# Autodesk Inventor assembly: shooter launcher
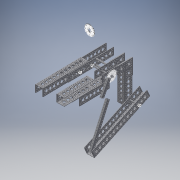
[picture p0: Inventor's stored thumbnail of the model, 180x180]
Saved by Autodesk Inventor 2017 (Build 210142000, 142)
## iProperties
Created: 2018-05-23
Part Number: shooter launcher
Document SubType Name: Assembly
Designer: User
Author: User
## Documents named in this file (16)
- C:\Robotics\CAD\2018-19_CAD\Offseason\shooter launcher.iam
- catapalt ball shoote.iam
- C:\Robotics\CAD\COTSParts\Actobotics\585 parts\585446Channel6in.ipt
- C:\Robotics\CAD\COTSParts\Actobotics\585 parts\585628FlatPattern90degreesA.ipt
- C:\Robotics\CAD\COTSParts\Tetrix\Hex standoff 2in.ipt
- C:\Robotics\CAD\COTSParts\Actobotics\615 parts\615106Sprocket.5inBore.25inPitch24Teeth.ipt
- C:\Robotics\CAD\COTSParts\Actobotics\535 parts\535198Bearing.25ID.5OD.ipt
- C:\Robotics\CAD\COTSParts\Actobotics\Collar.ipt
- C:\Robotics\CAD\COTSParts\Actobotics\585 parts\585450Channel9in.ipt
- C:\Robotics\CAD\COTSParts\Actobotics\585 parts\585454Channel12in.ipt
- C:\Robotics\CAD\COTSParts\Actobotics\634 parts\634080.25inDShaft4inLong.ipt
- C:\Robotics\CAD\COTSParts\Fasteners\Nylon spacer .25.ipt
- C:\Robotics\CAD\COTSParts\Actobotics\545 parts\545618 clamping hub.ipt
- C:\Robotics\CAD\COTSParts\Actobotics\634 parts\634082.25inDShaft6inLong.ipt
- C:\Robotics\CAD\COTSParts\Actobotics\585 parts\585396MiniChannel8in.ipt
- C:\Robotics\CAD\COTSParts\Actobotics\585 parts\585382MiniChannel3in.ipt
## Components (33 placed, 14 different names)
1. 585446Channel6in:1 — Mate:1, Flush:1, Flush:2, Mate:2, Flush:4, Mate:3, Flush:6, Insert:1, Mate:10, Mate:11, Mate:12, Mate:13, Mate:14, Insert:9, Flush:7, Insert:11, Mate:57
2. 585446Channel6in:2 — Mate:1, Flush:1, Flush:2, Flush:3, Flush:5, Mate:26, Mate:27, Mate:28, Mate:29
3. 585628FlatPattern90degreesA:1 — Mate:3, Flush:5, Flush:6
4. 585628FlatPattern90degreesA:2 — Mate:2, Flush:3, Flush:4
5. Hex standoff 2in:1 — Insert:11
6. Hex standoff 2in:3 — Insert:1, Mate:25
7. 615106Sprocket.5inBore.25inPitch24Teeth:1 — Mate:58, Mate:59, Mate:60, Mate:61
8. 615106Sprocket.5inBore.25inPitch24Teeth:2
9. 535198Bearing.25ID.5OD:1 — Insert:10, Mate:21
10. 535198Bearing.25ID.5OD:2 — Mate:12, Mate:13
11. 535198Bearing.25ID.5OD:3 — Mate:10, Mate:11, Insert:6
12. 535198Bearing.25ID.5OD:4 — Insert:8, Mate:23, Mate:54
13. Collar:1 — Insert:6, Mate:20
14. Collar:3 — Mate:21, Mate:55
15. Collar:4 — Insert:8, Mate:53, Flush:11
16. 585446Channel6in:3 — Mate:14, Insert:9, Flush:7, Mate:15, Flush:8, Mate:16
17. 585446Channel6in:4 — Mate:15, Flush:8, Mate:16, Flush:9
18. 585450Channel9in:1 — Mate:17, Mate:19, Mate:20, Insert:10, Mate:23, Flush:9, Mate:24, Mate:25, Mate:54
19. 585450Channel9in:2 — Mate:17, Mate:19, Mate:24
20. 585454Channel12in:1 — Mate:30, Mate:38, Mate:49, Insert:12
21. 634080.25inDShaft4inLong:1 — Mate:39, Mate:40, Mate:44, Mate:46, Mate:51, Flush:10
22. 535198Bearing.25ID.5OD:5 — Mate:38, Mate:48, Mate:51
23. 535198Bearing.25ID.5OD:6 — Mate:28, Mate:29, Mate:52
24. 535198Bearing.25ID.5OD:7 — Mate:30, Mate:40, Mate:49, Mate:50
25. 535198Bearing.25ID.5OD:8 — Mate:26, Mate:27, Mate:35, Mate:47
26. Collar:5 — Mate:35, Mate:39, Mate:50, Flush:10
27. Collar:6 — Mate:44, Mate:52
28. Nylon spacer .25:1 — Mate:46, Mate:47, Mate:48
29. Collar:7
30. 545618 clamping hub:1 — Mate:56, Mate:57, Mate:58, Mate:59, Mate:60
31. 634082.25inDShaft6inLong:1 — Mate:53, Mate:55, Mate:56, Flush:11
32. 585396MiniChannel8in:1 — Insert:12, Mate:62
33. 585382MiniChannel3in:1 — Mate:61, Mate:62
## Relationships (62: Mate 44, Flush 11, Insert 7)
- Mate:1: 585446Channel6in:1 ↔ 585446Channel6in:2
- Flush:1: 585446Channel6in:1 ↔ 585446Channel6in:2
- Flush:2: 585446Channel6in:1 ↔ 585446Channel6in:2
- Mate:2: 585446Channel6in:1 ↔ 585628FlatPattern90degreesA:2
- Flush:3: 585446Channel6in:2 ↔ 585628FlatPattern90degreesA:2
- Flush:4: 585446Channel6in:1 ↔ 585628FlatPattern90degreesA:2
- Mate:3: 585446Channel6in:1 ↔ 585628FlatPattern90degreesA:1
- Flush:5: 585446Channel6in:2 ↔ 585628FlatPattern90degreesA:1
- Flush:6: 585446Channel6in:1 ↔ 585628FlatPattern90degreesA:1
- Insert:1: 585446Channel6in:1 ↔ Hex standoff 2in:3
- Mate:10: 585446Channel6in:1 ↔ 535198Bearing.25ID.5OD:3
- Mate:11: 585446Channel6in:1 ↔ 535198Bearing.25ID.5OD:3
- Mate:12: 585446Channel6in:1 ↔ 535198Bearing.25ID.5OD:2
- Mate:13: 585446Channel6in:1 ↔ 535198Bearing.25ID.5OD:2
- Insert:6: 535198Bearing.25ID.5OD:3 ↔ Collar:1
- Insert:8: 535198Bearing.25ID.5OD:4 ↔ Collar:4
- Mate:14: 585446Channel6in:1 ↔ 585446Channel6in:3
- Insert:9: 585446Channel6in:1 ↔ 585446Channel6in:3
- Flush:7: 585446Channel6in:1 ↔ 585446Channel6in:3
- Mate:15: 585446Channel6in:3 ↔ 585446Channel6in:4
- Flush:8: 585446Channel6in:3 ↔ 585446Channel6in:4
- Mate:16: 585446Channel6in:3 ↔ 585446Channel6in:4
- Mate:17: 585450Channel9in:1 ↔ 585450Channel9in:2
- Mate:19 (-101.6 mm): 585450Channel9in:1 ↔ 585450Channel9in:2
- Mate:20: Collar:1 ↔ 585450Channel9in:1
- Insert:10: 535198Bearing.25ID.5OD:1 ↔ 585450Channel9in:1
- Mate:21: 535198Bearing.25ID.5OD:1 ↔ Collar:3
- Mate:23: 535198Bearing.25ID.5OD:4 ↔ 585450Channel9in:1
- Flush:9: 585446Channel6in:4 ↔ 585450Channel9in:1
- Mate:24: 585450Channel9in:1 ↔ 585450Channel9in:2
- Insert:11: 585446Channel6in:1 ↔ Hex standoff 2in:1
- Mate:25: Hex standoff 2in:3 ↔ 585450Channel9in:1
- Mate:26: 585446Channel6in:2 ↔ 535198Bearing.25ID.5OD:8
- Mate:27: 585446Channel6in:2 ↔ 535198Bearing.25ID.5OD:8
- Mate:28: 585446Channel6in:2 ↔ 535198Bearing.25ID.5OD:6
- Mate:29: 585446Channel6in:2 ↔ 535198Bearing.25ID.5OD:6
- Mate:30: 585454Channel12in:1 ↔ 535198Bearing.25ID.5OD:7
- Mate:35: 535198Bearing.25ID.5OD:8 ↔ Collar:5
- Mate:38: 585454Channel12in:1 ↔ 535198Bearing.25ID.5OD:5
- Mate:39: 634080.25inDShaft4inLong:1 ↔ Collar:5
- Mate:40: 634080.25inDShaft4inLong:1 ↔ 535198Bearing.25ID.5OD:7
- Mate:44: 634080.25inDShaft4inLong:1 ↔ Collar:6
- Mate:46: 634080.25inDShaft4inLong:1 ↔ Nylon spacer .25:1
- Mate:47: 535198Bearing.25ID.5OD:8 ↔ Nylon spacer .25:1
- Mate:48: 535198Bearing.25ID.5OD:5 ↔ Nylon spacer .25:1
- Mate:49: 585454Channel12in:1 ↔ 535198Bearing.25ID.5OD:7
- Mate:50: 535198Bearing.25ID.5OD:7 ↔ Collar:5
- Mate:51: 634080.25inDShaft4inLong:1 ↔ 535198Bearing.25ID.5OD:5
- Mate:52: 535198Bearing.25ID.5OD:6 ↔ Collar:6
- Flush:10 (0.6858 mm): 634080.25inDShaft4inLong:1 ↔ Collar:5
- Mate:53: Collar:4 ↔ 634082.25inDShaft6inLong:1
- Mate:54: 535198Bearing.25ID.5OD:4 ↔ 585450Channel9in:1
- Mate:55: Collar:3 ↔ 634082.25inDShaft6inLong:1
- Mate:56: 545618 clamping hub:1 ↔ 634082.25inDShaft6inLong:1
- Flush:11: Collar:4 ↔ 634082.25inDShaft6inLong:1
- Mate:57: 585446Channel6in:1 ↔ 545618 clamping hub:1
- Mate:58: 615106Sprocket.5inBore.25inPitch24Teeth:1 ↔ 545618 clamping hub:1
- Mate:59: 615106Sprocket.5inBore.25inPitch24Teeth:1 ↔ 545618 clamping hub:1
- Mate:60: 615106Sprocket.5inBore.25inPitch24Teeth:1 ↔ 545618 clamping hub:1
- Insert:12: 585454Channel12in:1 ↔ 585396MiniChannel8in:1
- Mate:61: 615106Sprocket.5inBore.25inPitch24Teeth:1 ↔ 585382MiniChannel3in:1
- Mate:62: 585396MiniChannel8in:1 ↔ 585382MiniChannel3in:1
